# Autodesk Inventor assembly: terminal_front
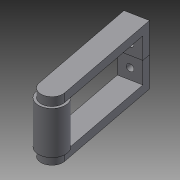
[picture p0: Inventor's stored thumbnail of the model, 180x180]
Saved by Autodesk Inventor 2018 (Build 220112000, 112)
## iProperties
Created: 2017-06-03
Part Number: terminal_front
Document SubType Name: Assembly
Designer: AYUSH SHUKLA
Author: AYUSH SHUKLA
## Documents named in this file (3)
- C:\Study\BTP2\Robomuse Inventor CAD\terminal_front.iam
- C:\Study\BTP2\Robomuse Inventor CAD\terminal_front.ipt
- C:\Study\BTP2\Robomuse Inventor CAD\terminal_mount_front.ipt
## Components (3 placed, 2 different names)
1. terminal_front:1 — Mate:1, Mate:2, Mate:3
2. terminal_mount_front:1 — Mate:1, Mate:2, Mate:4, Flush:1
3. terminal_mount_front:2 — Mate:3, Mate:4, Flush:1
## Relationships (5: Mate 4, Flush 1)
- Mate:1: terminal_front:1 ↔ terminal_mount_front:1
- Mate:2: terminal_front:1 ↔ terminal_mount_front:1
- Mate:3: terminal_front:1 ↔ terminal_mount_front:2
- Mate:4: terminal_mount_front:1 ↔ terminal_mount_front:2
- Flush:1: terminal_mount_front:1 ↔ terminal_mount_front:2
